# Autodesk Inventor assembly: S24x2
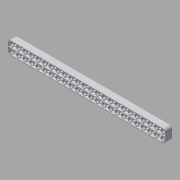
[picture p0: Inventor's stored thumbnail of the model, 180x180]
Saved by Autodesk Inventor 2019.3 (Build 233278000, 278)
## iProperties
Created: 2019-01-31
Part Number: S24x2
Document SubType Name: Assembly
Designer: Varga Daniel
Author: Varga Daniel
## Documents named in this file (11)
- C:\!_Dani\!_cloud\OneDrive\!_munka\Revolution\RevvyDemoKit\Structural parts\Beams\Straight Beams\S2+x2.iam
- C:\!_Dani\!_cloud\OneDrive\!_munka\Revolution\RevvyDemoKit\Structural parts\Beams\beam_corner_part.ipt
- C:\!_Dani\!_cloud\OneDrive\!_munka\Revolution\RevvyDemoKit\Structural parts\Beams\beam_side_part.ipt
- S12x2.iam
- S16x2.iam
- S24x2.iam
- S2x2.iam
- S3x2.iam
- S4x2.iam
- S6x2.iam
- S8x2.iam
## Components (48 placed, 2 different names)
1. beam_corner_part:1 — Flush:1, Flush:2, Mate:1, Flush:7, Mate:4, Flush:8, Flush:9, Mate:5, Flush:10
2. beam_corner_part:2 — Flush:1, Flush:2, Mate:1
3. beam_corner_part:3 — Flush:5, Flush:6, Mate:3, Flush:7, Mate:4, Flush:10
4. beam_corner_part:4 — Flush:5, Flush:6, Mate:3
5. beam_side_part:1 — Mate:2, Flush:3, Flush:4, Flush:8, Flush:9, Mate:5
6. beam_side_part:2 — Mate:2, Flush:3, Flush:4
7. beam_side_part:3
8. beam_side_part:4
9. beam_side_part:5
10. beam_side_part:6
11. beam_side_part:7
12. beam_side_part:8
13. beam_side_part:9
14. beam_side_part:10
15. beam_side_part:11
16. beam_side_part:12
17. beam_side_part:13
18. beam_side_part:14
19. beam_side_part:15
20. beam_side_part:16
21. beam_side_part:17
22. beam_side_part:18
23. beam_side_part:19
24. beam_side_part:20
25. beam_side_part:21
26. beam_side_part:22
27. beam_side_part:23
28. beam_side_part:24
29. beam_side_part:25
30. beam_side_part:26
31. beam_side_part:27
32. beam_side_part:28
33. beam_side_part:29
34. beam_side_part:30
35. beam_side_part:31
36. beam_side_part:32
37. beam_side_part:33
38. beam_side_part:34
39. beam_side_part:35
40. beam_side_part:36
41. beam_side_part:37
42. beam_side_part:38
43. beam_side_part:39
44. beam_side_part:40
45. beam_side_part:41
46. beam_side_part:42
47. beam_side_part:43
48. beam_side_part:44
## Component patterns: (22 elements, first: beam_side_part:1 + beam_side_part:2)
## Relationships (15: Flush 10, Mate 5)
- Flush:1: beam_corner_part:1 ↔ beam_corner_part:2
- Flush:2: beam_corner_part:1 ↔ beam_corner_part:2
- Mate:1: beam_corner_part:1 ↔ beam_corner_part:2
- Mate:2: beam_side_part:1 ↔ beam_side_part:2
- Flush:3: beam_side_part:1 ↔ beam_side_part:2
- Flush:4: beam_side_part:1 ↔ beam_side_part:2
- Flush:5: beam_corner_part:3 ↔ beam_corner_part:4
- Flush:6: beam_corner_part:3 ↔ beam_corner_part:4
- Mate:3: beam_corner_part:3 ↔ beam_corner_part:4
- Flush:7: beam_corner_part:1 ↔ beam_corner_part:3
- Mate:4 (220 mm): beam_corner_part:1 ↔ beam_corner_part:3
- Flush:8: beam_corner_part:1 ↔ beam_side_part:1
- Flush:9: beam_corner_part:1 ↔ beam_side_part:1
- Mate:5: beam_corner_part:1 ↔ beam_side_part:1
- Flush:10: beam_corner_part:1 ↔ beam_corner_part:3
